# Autodesk Inventor assembly: Zusammenbau
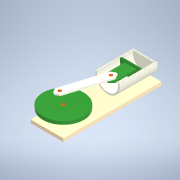
[picture p0: Inventor's stored thumbnail of the model, 180x180]
Saved by Autodesk Inventor 2022 (Build 260153000, 153)
## iProperties
Created: 2022-06-01
Part Number: Zusammenbau
Document SubType Name: Assembly
Designer: kaebi
Author: kaebi
## Documents named in this file (8)
- C:\Users\kaebi\OneDrive - mci4me.at\03_MCI Master\4.Semester_SS2022\Masterarbeit\Software\CAD\1_FormatTesting\Zusammenbau.iam
- C:\Users\kaebi\OneDrive - mci4me.at\03_MCI Master\4.Semester_SS2022\Masterarbeit\Software\CAD\1_FormatTesting\Grundplatte.ipt
- C:\Users\kaebi\OneDrive - mci4me.at\03_MCI Master\4.Semester_SS2022\Masterarbeit\Software\CAD\1_FormatTesting\Bolzen.ipt
- C:\Users\kaebi\OneDrive - mci4me.at\03_MCI Master\4.Semester_SS2022\Masterarbeit\Software\CAD\1_FormatTesting\Schwingscheibe.ipt
- C:\Users\kaebi\OneDrive - mci4me.at\03_MCI Master\4.Semester_SS2022\Masterarbeit\Software\CAD\1_FormatTesting\Hulse.ipt
- C:\Users\kaebi\OneDrive - mci4me.at\03_MCI Master\4.Semester_SS2022\Masterarbeit\Software\CAD\1_FormatTesting\Deckel.ipt
- C:\Users\kaebi\OneDrive - mci4me.at\03_MCI Master\4.Semester_SS2022\Masterarbeit\Software\CAD\1_FormatTesting\Schenkel.ipt
- C:\Users\kaebi\OneDrive - mci4me.at\03_MCI Master\4.Semester_SS2022\Masterarbeit\Software\CAD\1_FormatTesting\BolzenKlein.ipt
## Components (8 placed, 7 different names)
1. Grundplatte:1 — Passend:1, Passend:2, Passend:3, Passend:4, Fluchtend:1, Passend:6, Tangential:1, Fluchtend:3, Winkel:1
2. Bolzen:1 — Passend:4, Fluchtend:1, Passend:5, Fluchtend:2
3. Schwingscheibe:1 — Passend:5, Fluchtend:2, Passend:8, Passend:10
4. Hulse:1 — Passend:6, Tangential:1, Fluchtend:3, Passend:7
5. Deckel:1 — Passend:7, Winkel:1, Passend:9
6. Schenkel:1 — Passend:8, Passend:9, Passend:10, Passend:11, Fluchtend:4, Passend:12, Fluchtend:5
7. BolzenKlein:1 — Passend:12, Fluchtend:5
8. BolzenKlein:2 — Passend:11, Fluchtend:4
## Relationships (19: Mate 12, Flush 5, Tangent 1, Angle 1)
- Passend:1 [Mate]: Grundplatte:1
- Passend:2 [Mate]: Grundplatte:1
- Passend:3 [Mate]: Grundplatte:1
- Passend:4 [Mate]: Grundplatte:1 ↔ Bolzen:1
- Fluchtend:1 [Flush]: Grundplatte:1 ↔ Bolzen:1
- Passend:5 [Mate]: Bolzen:1 ↔ Schwingscheibe:1
- Fluchtend:2 [Flush]: Bolzen:1 ↔ Schwingscheibe:1
- Passend:6 [Mate]: Grundplatte:1 ↔ Hulse:1
- Tangential:1: Grundplatte:1 ↔ Hulse:1
- Fluchtend:3 [Flush]: Grundplatte:1 ↔ Hulse:1
- Passend:7 [Mate]: Hulse:1 ↔ Deckel:1
- Winkel:1 [Angle] (0 deg): Grundplatte:1 ↔ Deckel:1
- Passend:8 [Mate]: Schwingscheibe:1 ↔ Schenkel:1
- Passend:9 [Mate]: Deckel:1 ↔ Schenkel:1
- Passend:10 [Mate]: Schwingscheibe:1 ↔ Schenkel:1
- Passend:11 [Mate]: Schenkel:1 ↔ BolzenKlein:2
- Fluchtend:4 [Flush]: Schenkel:1 ↔ BolzenKlein:2
- Passend:12 [Mate]: Schenkel:1 ↔ BolzenKlein:1
- Fluchtend:5 [Flush]: Schenkel:1 ↔ BolzenKlein:1
